# Autodesk Inventor assembly: Ensamble del Arreglo
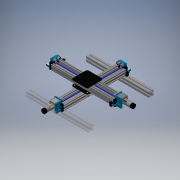
[picture p0: Inventor's stored thumbnail of the model, 180x180]
Saved by Autodesk Inventor 2018.3 (Build 223284000, 284)
## iProperties
Created: 2020-12-03
Part Number: Ensamble del Arreglo
Material: Genérico
Description: STEP AP203
Document SubType Name: Assembly
Designer: SERGIO ROMO
Sending System: SolidWorks 2019
Preprocessor: SwSTEP 2.0
Title: Ensamble del Arreglo.STEP
Revision Number: ANY
## Documents named in this file (13)
- C:\Users\SERGIO ROMO\Documents\GitHub\RemBot\CAD\Balanceo de masa\Inventor\Ensamble del Arreglo.iam
- C:\Users\SERGIO ROMO\Documents\GitHub\RemBot\CAD\Balanceo de masa\Inventor\C-Beam Actuator Lineal 500mm (Sin motor, sin carrito).ipt
- C:\Users\SERGIO ROMO\Documents\GitHub\RemBot\CAD\Balanceo de masa\Inventor\XLarge C-Beam Gantry Kit.iam
- C:\Users\SERGIO ROMO\Documents\GitHub\RemBot\CAD\Balanceo de masa\Inventor\Perfil de Aluminio.ipt
- C:\Users\SERGIO ROMO\Documents\GitHub\RemBot\CAD\Balanceo de masa\Inventor\Tubito.ipt
- C:\Users\SERGIO ROMO\Documents\GitHub\RemBot\CAD\Balanceo de masa\Inventor\Clavo.ipt
- C:\Users\SERGIO ROMO\Documents\GitHub\RemBot\CAD\Balanceo de masa\Inventor\Gearmotor_37D_19a1.ipt
- C:\Users\SERGIO ROMO\Documents\GitHub\RemBot\CAD\Balanceo de masa\Inventor\Impresion3D.ipt
- C:\Users\SERGIO ROMO\Documents\GitHub\RemBot\CAD\Balanceo de masa\Inventor\C-Beam Gantry Plate XLarge.step.ipt
- C:\Users\SERGIO ROMO\Documents\GitHub\RemBot\CAD\Balanceo de masa\Inventor\Bracket Inventor.ipt
- C:\Users\SERGIO ROMO\Documents\GitHub\RemBot\CAD\Balanceo de masa\Inventor\KW8-2.ipt
- C:\Users\SERGIO ROMO\Documents\GitHub\RemBot\CAD\Balanceo de masa\Inventor\HC-SR04 Ultrasonico.iam
- C:\Users\SERGIO ROMO\Documents\GitHub\RemBot\CAD\Balanceo de masa\Inventor\Impresion3D sin el bracket.ipt
## Components (26 placed, 18 different names)
1. C-Beam Actuator Lineal 500mm (Sin motor, sin carrito)_1 — De rotación:2
2. XLarge C-Beam Gantry Kit_2 [sub-assembly] — Rígido:1
3. Perfil de Aluminio_4
4. Perfil de Aluminio_5
5. Tubito_6
6. Tubito_7
7. Clavo_8
8. Clavo_9
9. Gearmotor_37D_19a1_10
10. Gearmotor_37D_19a1_22
11. Impresion3D_28 — Coincidencia:1, Coincidencia:4, De rotación:1
12. C-Beam Actuator Lineal 500mm (Sin motor, sin carrito):2 — Rígido:1, Coincidencia:2
13. C-Beam Gantry Plate XLarge.step:1
14. Bracket Inventor:1 — Coincidencia:1
15. Bracket Inventor:2 — Coincidencia:3
16. Impresion3D:2 — Coincidencia:2, Coincidencia:3, Coincidencia:5
17. KW8-2:1 — Coincidencia:4
18. HC-SR04 Ultrasonico:1 [sub-assembly] — De rotación:1
19. HC-SR04 Ultrasonico:2 [sub-assembly]
20. KW8-2:2 — Coincidencia:5
21. KW8-2:3
22. HC-SR04 Ultrasonico:3 [sub-assembly]
23. KW8-2:4
24. HC-SR04 Ultrasonico:4 [sub-assembly]
25. Impresion3D sin el bracket:1 — De rotación:2
26. Impresion3D sin el bracket:2
## Relationships (8: Mate 5, RevoluteJoint 2, WeldJoint 1)
- Rígido:1 [WeldJoint]: XLarge C-Beam Gantry Kit_2 ↔ C-Beam Actuator Lineal 500mm (Sin motor, sin carrito):2
- Coincidencia:1 [Mate]: Impresion3D_28 ↔ Bracket Inventor:1
- Coincidencia:2 [Mate]: C-Beam Actuator Lineal 500mm (Sin motor, sin carrito):2 ↔ Impresion3D:2
- Coincidencia:3 [Mate]: Bracket Inventor:2 ↔ Impresion3D:2
- Coincidencia:4 [Mate]: Impresion3D_28 ↔ KW8-2:1
- Coincidencia:5 [Mate]: Impresion3D:2 ↔ KW8-2:2
- De rotación:1 [RevoluteJoint]: Impresion3D_28 ↔ HC-SR04 Ultrasonico:1
- De rotación:2 [RevoluteJoint]: C-Beam Actuator Lineal 500mm (Sin motor, sin carrito)_1 ↔ Impresion3D sin el bracket:1
